# Autodesk Inventor assembly: frame assembly 9
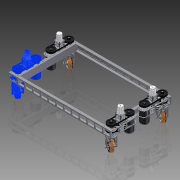
[picture p0: Inventor's stored thumbnail of the model, 180x180]
Saved by Autodesk Inventor 2012 (Build 160160000, 160)
## iProperties
Created: 2013-11-05
Part Number: frame assembly 9
Document SubType Name: Assembly
Designer: Bryce
Author: Bryce
## Documents named in this file (4)
- C:\Users\Bryce\Dropbox\Inventor Design Project Files\Independent Swerves\Inventor 2012\frame assembly 9.iam
- C:\Users\Bryce\Dropbox\Inventor Design Project Files\Independent Swerves\Inventor 2012\FULL SWERVE DRIVE ASSEMBLY!  6!.iam
- C:\Users\Bryce\Dropbox\Inventor Design Project Files\Independent Swerves\Inventor 2012\2.25 U frame 2.ipt
- C:\Users\Bryce\Dropbox\Inventor Design Project Files\Independent Swerves\Inventor 2012\2.25 U frame front.ipt
## Components (8 placed, 3 different names)
1. FULL SWERVE DRIVE ASSEMBLY!  6!:1 [sub-assembly] — Flush:1, Flush:2, Flush:3, Flush:5, Mate:1, Mate:2, Flush:9, Mate:5, Mate:6, Mate:7, Mate:8, Flush:10
2. FULL SWERVE DRIVE ASSEMBLY!  6!:2 [sub-assembly] — Flush:3, Flush:5, Flush:7, Mate:2, Mate:3, Mate:4, Flush:8
3. FULL SWERVE DRIVE ASSEMBLY!  6!:3 [sub-assembly] — Flush:4, Flush:6, Flush:7
4. FULL SWERVE DRIVE ASSEMBLY!  6!:4 [sub-assembly] — Flush:1, Flush:2, Flush:4, Flush:6, Mate:1, Mate:9, Flush:11, Mate:10
5. 2.25 U frame 2:1 — Mate:3, Mate:4, Flush:8
6. 2.25 U frame 2:2 — Flush:9, Mate:5, Mate:6
7. 2.25 U frame front:1 — Mate:9, Flush:11, Mate:10
8. 2.25 U frame front:2 — Mate:7, Mate:8, Flush:10
## Relationships (21: Flush 11, Mate 10)
- Flush:1: FULL SWERVE DRIVE ASSEMBLY!  6!:1 ↔ FULL SWERVE DRIVE ASSEMBLY!  6!:4
- Flush:2: FULL SWERVE DRIVE ASSEMBLY!  6!:1 ↔ FULL SWERVE DRIVE ASSEMBLY!  6!:4
- Flush:3: FULL SWERVE DRIVE ASSEMBLY!  6!:1 ↔ FULL SWERVE DRIVE ASSEMBLY!  6!:2
- Flush:4: FULL SWERVE DRIVE ASSEMBLY!  6!:3 ↔ FULL SWERVE DRIVE ASSEMBLY!  6!:4
- Flush:5: FULL SWERVE DRIVE ASSEMBLY!  6!:1 ↔ FULL SWERVE DRIVE ASSEMBLY!  6!:2
- Flush:6: FULL SWERVE DRIVE ASSEMBLY!  6!:3 ↔ FULL SWERVE DRIVE ASSEMBLY!  6!:4
- Flush:7: FULL SWERVE DRIVE ASSEMBLY!  6!:2 ↔ FULL SWERVE DRIVE ASSEMBLY!  6!:3
- Mate:1 (-520.7 mm): FULL SWERVE DRIVE ASSEMBLY!  6!:1 ↔ FULL SWERVE DRIVE ASSEMBLY!  6!:4
- Mate:2 (-889 mm): FULL SWERVE DRIVE ASSEMBLY!  6!:1 ↔ FULL SWERVE DRIVE ASSEMBLY!  6!:2
- Mate:3: FULL SWERVE DRIVE ASSEMBLY!  6!:2 ↔ 2.25 U frame 2:1
- Mate:4: FULL SWERVE DRIVE ASSEMBLY!  6!:2 ↔ 2.25 U frame 2:1
- Flush:8: FULL SWERVE DRIVE ASSEMBLY!  6!:2 ↔ 2.25 U frame 2:1
- Flush:9: FULL SWERVE DRIVE ASSEMBLY!  6!:1 ↔ 2.25 U frame 2:2
- Mate:5: FULL SWERVE DRIVE ASSEMBLY!  6!:1 ↔ 2.25 U frame 2:2
- Mate:6: FULL SWERVE DRIVE ASSEMBLY!  6!:1 ↔ 2.25 U frame 2:2
- Mate:7: FULL SWERVE DRIVE ASSEMBLY!  6!:1 ↔ 2.25 U frame front:2
- Mate:8: FULL SWERVE DRIVE ASSEMBLY!  6!:1 ↔ 2.25 U frame front:2
- Flush:10: FULL SWERVE DRIVE ASSEMBLY!  6!:1 ↔ 2.25 U frame front:2
- Mate:9: FULL SWERVE DRIVE ASSEMBLY!  6!:4 ↔ 2.25 U frame front:1
- Flush:11: FULL SWERVE DRIVE ASSEMBLY!  6!:4 ↔ 2.25 U frame front:1
- Mate:10: FULL SWERVE DRIVE ASSEMBLY!  6!:4 ↔ 2.25 U frame front:1
